# Autodesk Inventor assembly: FemaleHeader
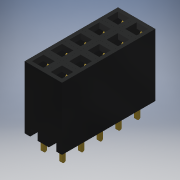
[picture p0: Inventor's stored thumbnail of the model, 180x180]
Saved by Autodesk Inventor 2018 (Build 220112000, 112)
## iProperties
Created: 2013-05-21
Part Number: FemaleHeader
Document SubType Name: Assembly
Designer: dkt01
Sending System: SolidWorks 2012
Last Author: simonx
Last Saved: 2013-05-21
pinx: 2.000 ul
piny: 5.000 ul
Author: dkt01
## Documents named in this file (2)
- C:\Users\dktur\Dropbox\StackLightMonitor\CAD\FemaleHeader.iam
- C:\Users\dktur\Dropbox\StackLightMonitor\CAD\FemaleHeader_Single.iam
## Components (10 placed, 2 different names)
1. header:1 [sub-assembly]
2. FemaleHeader_Single:5 [sub-assembly]
3. FemaleHeader_Single:6 [sub-assembly]
4. FemaleHeader_Single:7 [sub-assembly]
5. FemaleHeader_Single:8 [sub-assembly]
6. FemaleHeader_Single:9 [sub-assembly]
7. FemaleHeader_Single:10 [sub-assembly]
8. FemaleHeader_Single:11 [sub-assembly]
9. FemaleHeader_Single:12 [sub-assembly]
10. FemaleHeader_Single:13 [sub-assembly]
## Component patterns: (10 elements, first: header:1)
